# Autodesk Inventor assembly: screw_lift
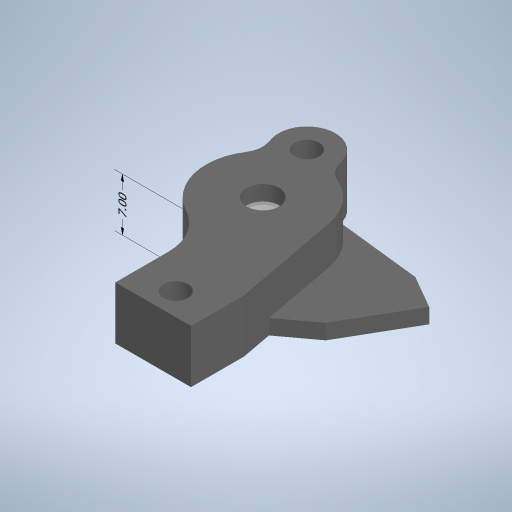
[picture p0: Inventor's stored thumbnail of the model, 512x512]
Saved by Autodesk Inventor 2024.1 (Build 281209000, 209)
## iProperties
Created: 2025-01-18
Part Number: screw_lift
Document SubType Name: Assembly
Designer: hibik
Author: hibik
## Documents named in this file (4)
- C:\Users\hibik\Documents\Robomech\RESCUE\ORCA\hard\fork\right\screw_lift.iam
- C:\Users\hibik\Documents\Robomech\RESCUE\ORCA\hard\std_parts\nat_M4.ipt
- C:\Users\hibik\Documents\Robomech\RESCUE\ORCA\hard\fork\right\screw_lift_under.ipt
- C:\Users\hibik\Documents\Robomech\RESCUE\ORCA\hard\fork\right\screw_lift_upper.ipt
## Components (3 placed, 3 different names)
1. nat_M4:1 — 挿入:1, 角度:1
2. screw_lift_under:1 — 挿入:1, 角度:1, フラッシュ:1, フラッシュ:2, メイト:1
3. screw_lift_upper:1 — フラッシュ:1, フラッシュ:2, メイト:1
## Relationships (5: Flush 2, Insert 1, Angle 1, Mate 1)
- 挿入:1 [Insert]: nat_M4:1 ↔ screw_lift_under:1
- 角度:1 [Angle] (0 deg): nat_M4:1 ↔ screw_lift_under:1
- フラッシュ:1 [Flush]: screw_lift_under:1 ↔ screw_lift_upper:1
- フラッシュ:2 [Flush]: screw_lift_under:1 ↔ screw_lift_upper:1
- メイト:1 [Mate]: screw_lift_under:1 ↔ screw_lift_upper:1
